# Autodesk Inventor assembly: CanSat
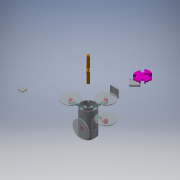
[picture p0: Inventor's stored thumbnail of the model, 180x180]
Saved by Autodesk Inventor 2018 (Build 220112000, 112)
## iProperties
Created: 2017-12-31
Part Number: CanSat
Document SubType Name: Assembly
Designer: suchanek
Author: suchanek
## Documents named in this file (17)
- C:\Users\Suchanek\Programming\CanSat\Schematics\Model\CanSat.iam
- C:\Users\Suchanek\Programming\CanSat\Schematics\Model\Hull.ipt
- C:\Users\Suchanek\Programming\CanSat\Schematics\Model\Arm.ipt
- C:\Users\Suchanek\Programming\CanSat\Schematics\Model\Motor.ipt
- C:\Users\Suchanek\Programming\CanSat\Schematics\Model\Rotor.ipt
- C:\Users\Suchanek\Programming\CanSat\Schematics\Model\Servo.ipt
- C:\Users\Suchanek\Programming\CanSat\Schematics\Model\Spring.ipt
- C:\Users\Suchanek\Programming\CanSat\Schematics\Model\Servo_bit.ipt
- C:\Users\Suchanek\Programming\CanSat\Schematics\Model\Scraper.ipt
- C:\Users\Suchanek\Programming\CanSat\Schematics\Model\Petri.ipt
- C:\Users\Suchanek\Programming\CanSat\Schematics\Model\Circuit.ipt
- C:\Users\Suchanek\Programming\CanSat\Schematics\Model\Flight_controler.ipt
- C:\Users\Suchanek\Programming\CanSat\Schematics\Model\HGLRC Micro 13A 4in1 BLHeli_S.ipt
- C:\Users\Suchanek\Programming\CanSat\Schematics\Model\SIM808 Module GSM GPRS GPS Breakout Board SIM808 for Arduino Raspberry.ipt
- C:\Users\Suchanek\Programming\CanSat\Schematics\Model\Motor_holder.ipt
- C:\Users\Suchanek\Programming\CanSat\Schematics\Model\Battery.ipt
- C:\Users\Suchanek\Programming\CanSat\Schematics\Model\Hull_bottom.ipt
## Components (31 placed, 16 different names)
1. Hull:1 — Flush:1, Slider:1, Planar:1, Rigid:9, Rotational:26, Rotational:27, Slider:2, Rotational:31, Rotational:32, Rotational:33, Planar:2, Mate:1, Mate:2
2. Arm:1 — Rigid:10, Rotational:31
3. Arm:2 — Rigid:12, Rotational:32
4. Arm:3 — Rigid:13, Rotational:33
5. Arm:4 — Rigid:11, Rotational:27
6. Motor:1 — Rotational:8, Rigid:17
7. Motor:2 — Rotational:9, Rigid:16
8. Motor:3 — Rotational:11, Rigid:15
9. Motor:4 — Rotational:10, Rigid:14
10. Rotor:1 — Rotational:8
11. Rotor:2 — Rotational:10
12. Rotor:3 — Rotational:9
13. Rotor:4 — Rotational:11
14. Servo:1 — Flush:1, Slider:1, Rotational:24
15. Spring:1 — Rigid:6, Rigid:7
16. Servo_bit:1 — Rotational:24, Rigid:6
17. Scraper:1 — Rigid:7
18. Petri:1 — Planar:1
19. Circuit:1
20. Flight_controler:1
21. HGLRC Micro 13A 4in1 BLHeli_S:2 — Rigid:9
22. SIM808 Module GSM GPRS GPS Breakout Board SIM808 for Arduino Raspberry:1 — Rotational:26
23. Motor_holder:1 — Rigid:11, Rigid:17
24. Motor_holder:2 — Rigid:10, Rigid:14
25. Motor_holder:3 — Rigid:12, Rigid:15
26. Motor_holder:4 — Rigid:13, Rigid:16
27. Battery:1 — Rigid:18, Slider:2
28. Battery:2 — Rigid:19, Rigid:20
29. Battery:3 — Rigid:20
30. Battery:4 — Rigid:18, Rigid:19
31. Hull_bottom:1 — Planar:2, Mate:1, Mate:2
## Relationships (31: WeldJoint 14, RevoluteJoint 10, TranslationJoint 2, PlanarJoint 2, Mate 2, Flush 1)
- Rotational:8 [RevoluteJoint]: Motor:1 ↔ Rotor:1
- Rotational:9 [RevoluteJoint]: Motor:2 ↔ Rotor:3
- Rotational:10 [RevoluteJoint]: Motor:4 ↔ Rotor:2
- Rotational:11 [RevoluteJoint]: Motor:3 ↔ Rotor:4
- Flush:1: Hull:1 ↔ Servo:1
- Slider:1 [TranslationJoint]: Hull:1 ↔ Servo:1
- Rotational:24 [RevoluteJoint]: Servo:1 ↔ Servo_bit:1
- Rigid:6 [WeldJoint]: Spring:1 ↔ Servo_bit:1
- Rigid:7 [WeldJoint]: Spring:1 ↔ Scraper:1
- Planar:1: Hull:1 ↔ Petri:1
- Rigid:9 [WeldJoint]: Hull:1 ↔ HGLRC Micro 13A 4in1 BLHeli_S:2
- Rotational:26 [RevoluteJoint]: Hull:1 ↔ SIM808 Module GSM GPRS GPS Breakout Board SIM808 for Arduino Raspberry:1
- Rigid:10 [WeldJoint]: Arm:1 ↔ Motor_holder:2
- Rigid:11 [WeldJoint]: Arm:4 ↔ Motor_holder:1
- Rigid:12 [WeldJoint]: Arm:2 ↔ Motor_holder:3
- Rigid:13 [WeldJoint]: Arm:3 ↔ Motor_holder:4
- Rigid:14 [WeldJoint]: Motor:4 ↔ Motor_holder:2
- Rigid:15 [WeldJoint]: Motor:3 ↔ Motor_holder:3
- Rigid:16 [WeldJoint]: Motor:2 ↔ Motor_holder:4
- Rigid:17 [WeldJoint]: Motor:1 ↔ Motor_holder:1
- Rotational:27 [RevoluteJoint]: Hull:1 ↔ Arm:4
- Rigid:18 [WeldJoint]: Battery:1 ↔ Battery:4
- Rigid:19 [WeldJoint]: Battery:2 ↔ Battery:4
- Rigid:20 [WeldJoint]: Battery:2 ↔ Battery:3
- Slider:2 [TranslationJoint]: Hull:1 ↔ Battery:1
- Rotational:31 [RevoluteJoint]: Hull:1 ↔ Arm:1
- Rotational:32 [RevoluteJoint]: Hull:1 ↔ Arm:2
- Rotational:33 [RevoluteJoint]: Hull:1 ↔ Arm:3
- Planar:2: Hull:1 ↔ Hull_bottom:1
- Mate:1: Hull:1 ↔ Hull_bottom:1
- Mate:2: Hull:1 ↔ Hull_bottom:1
